# Autodesk Inventor assembly: CIM Motor
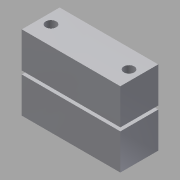
[picture p0: Inventor's stored thumbnail of the model, 180x180]
Saved by Autodesk Inventor 2013 (Build 170138000, 138)
## iProperties
Created: 2013-01-18
Part Number: CIM Motor
Document SubType Name: Assembly
Designer: Naphat
Author: Naphat
## Documents named in this file (2)
- C:\Users\carneeki\Desktop\Kiwi Robot\Imported Components\Motors\CIM Mount\CIM MotorCase.iam
- C:\Users\carneeki\Desktop\Kiwi Robot\Imported Components\Motors\CIM Mount\2.5 CIM mount.ipt
## Components (2 placed, 1 different names)
1. 2.5 CIM mount:1 — Insert:1, Insert:2
2. 2.5 CIM mount:2 — Insert:1, Insert:2
## Relationships (2: Insert 2)
- Insert:1 (4 mm): 2.5 CIM mount:1 ↔ 2.5 CIM mount:2
- Insert:2 (4 mm): 2.5 CIM mount:1 ↔ 2.5 CIM mount:2
